# Autodesk Inventor assembly: UQ205-topHolder-sample
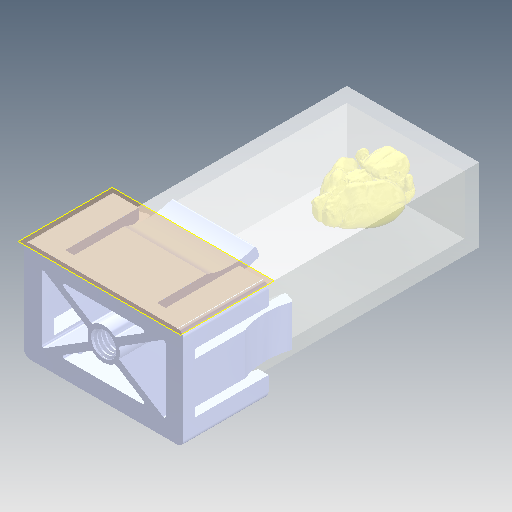
[picture p0: Inventor's stored thumbnail of the model, 512x512]
Saved by Autodesk Inventor 2021 (Build 250183000, 183)
## iProperties
Created: 2023-02-10
Part Number: UQ205-topHolder-sample
Document SubType Name: Assembly
Designer: nvladi
Author: nvladi
## Documents named in this file (4)
- C:\Users\Public\GitHub-public\benchtop-hardware\Benchtop\custom-parts\sample_handling\assemblies\UQ205-topHolder-sample.iam
- C:\Users\Public\GitHub-public\benchtop-hardware\Benchtop\custom-parts\sample_handling\cuvette-holders\Cuvette-22.5x12.5mm(UG205)\TopClamp-UG205_100943(Rechteck 2mm)_D.ipt
- C:\Users\Public\GitHub-public\benchtop-hardware\Benchtop\CAD-model-Inventor2021\library\Portmann Instruments\UQ-205-10x20x45mm.ipt
- C:\Users\Public\GitHub-public\benchtop-hardware\Benchtop\CAD-model-Inventor2021\library\samples\mousebrain2.ipt
## Components (3 placed, 3 different names)
1. TopClamp-UG205_100943(Rechteck 2mm)_D:1 — Mate:1, Flush:1, Flush:2
2. UQ-205-10x20x45mm:1 — Mate:1, Flush:1, Flush:2
3. mousebrain2:2
## Relationships (3: Flush 2, Mate 1)
- Mate:1: TopClamp-UG205_100943(Rechteck 2mm)_D:1 ↔ UQ-205-10x20x45mm:1
- Flush:1 (2.2 mm): TopClamp-UG205_100943(Rechteck 2mm)_D:1 ↔ UQ-205-10x20x45mm:1
- Flush:2 (-2.2 mm): TopClamp-UG205_100943(Rechteck 2mm)_D:1 ↔ UQ-205-10x20x45mm:1
